# Autodesk Inventor assembly: Assembly1
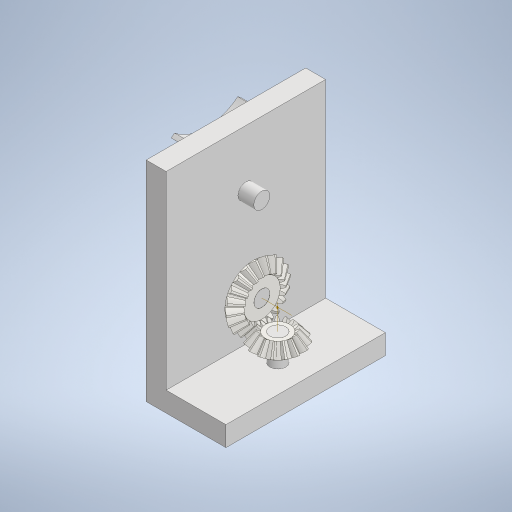
[picture p0: Inventor's stored thumbnail of the model, 512x512]
Saved by Autodesk Inventor 2023 (Build 270158000, 158)
## iProperties
Created: 2023-02-02
Part Number: Assembly1
Document SubType Name: Assembly
Designer: MOHIKA
Author: MOHIKA
## Documents named in this file (7)
- C:\Users\MOHIKA\Documents\Assembly1.iam
- C:\Users\MOHIKA\Documents\Support-plate.ipt
- C:\Users\MOHIKA\Documents\Geneva-driver.ipt
- C:\Users\MOHIKA\Documents\Geneva-driven.ipt
- C:\Users\MOHIKA\Documents\Shaft.ipt
- C:\Users\MOHIKA\Documents\Assembly1\Design Accelerator\Bevel Gears1.iam
- C:\Users\MOHIKA\Documents\Assembly1\Design Accelerator\Bevel Gears2.iam
## Components (8 placed, 5 different names)
1. Support-plate:1 — Mate:1, Mate:2, Mate:4, Mate:9
2. Geneva-driver:1 — Mate:1, Mate:2, Mate:3, Mate:7, Mate:8, Rotation:4
3. Geneva-driven:1 — Mate:3, Mate:4, Mate:5, Mate:6
4. Shaft:1 — Mate:7, Mate:8, Mate:10, Rotation:3, Rotation:4
5. Shaft:2 — Mate:9, Mate:11, Flush:1, Rotation:2
6. Shaft:3 — Mate:5, Mate:6
7. Bevel Gears:1 [sub-assembly] — Mate:10, Mate:12, Rotation:1, Rotation:3
8. Bevel Gears:2 [sub-assembly] — Mate:11, Mate:12, Flush:1, Rotation:1, Rotation:2
## Relationships (17: Mate 12, RelateRotation 4, Flush 1)
- Mate:1: Support-plate:1 ↔ Geneva-driver:1
- Mate:2: Support-plate:1 ↔ Geneva-driver:1
- Mate:3: Geneva-driver:1 ↔ Geneva-driven:1
- Mate:4: Support-plate:1 ↔ Geneva-driven:1
- Mate:5: Geneva-driven:1 ↔ Shaft:3
- Mate:6: Geneva-driven:1 ↔ Shaft:3
- Mate:7: Geneva-driver:1 ↔ Shaft:1
- Mate:8: Geneva-driver:1 ↔ Shaft:1
- Mate:9: Support-plate:1 ↔ Shaft:2
- Mate:10: Shaft:1 ↔ Bevel Gears:1
- Mate:11: Shaft:2 ↔ Bevel Gears:2
- Mate:12: Bevel Gears:1 ↔ Bevel Gears:2
- Flush:1: Shaft:2 ↔ Bevel Gears:2
- Rotation:1 [RelateRotation] (1.3333 ul): Bevel Gears:1 ↔ Bevel Gears:2
- Rotation:2 [RelateRotation] (1 ul): Shaft:2 ↔ Bevel Gears:2
- Rotation:3 [RelateRotation] (1 ul): Shaft:1 ↔ Bevel Gears:1
- Rotation:4 [RelateRotation] (1 ul): Geneva-driver:1 ↔ Shaft:1
